# Autodesk Inventor assembly: Super Gantry
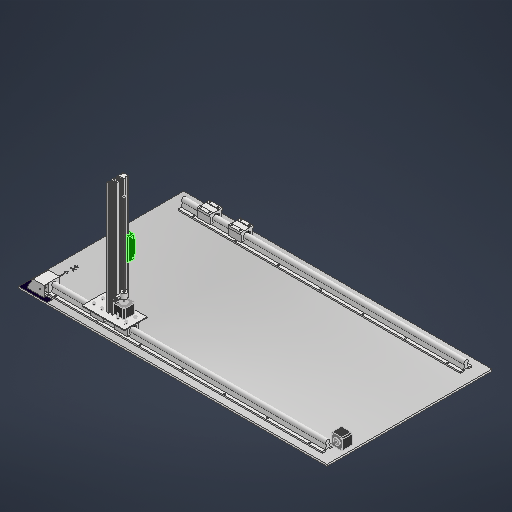
[picture p0: Inventor's stored thumbnail of the model, 512x512]
Saved by Autodesk Inventor 2025.1 (Build 291241000, 241)
## iProperties
Created: 2025-01-22
Part Number: Super Gantry
Document SubType Name: Assembly
Designer: jerem
Author: jerem
## Documents named in this file (3)
- C:\Users\jerem\Documents\GitHub\Perovskite-Automated-Synthesis-System\CAD\Gantry\Super Gantry.iam
- C:\Users\jerem\Documents\GitHub\Perovskite-Automated-Synthesis-System\CAD\Gantry\X Axis.iam
- C:\Users\jerem\Documents\GitHub\Perovskite-Automated-Synthesis-System\CAD\Gantry\Z Axis.iam
## Components (2 placed, 2 different names)
1. X Axis:1 [sub-assembly] — Mate:1, Mate:2, Mate:3, Mate:4, Mate:5
2. Z Axis:1 [sub-assembly] — Mate:1, Mate:2, Mate:3, Mate:4, Mate:5
## Relationships (5: Mate 5)
- Mate:1: X Axis:1 ↔ Z Axis:1
- Mate:2: X Axis:1 ↔ Z Axis:1
- Mate:3: X Axis:1 ↔ Z Axis:1
- Mate:4: X Axis:1 ↔ Z Axis:1
- Mate:5: X Axis:1 ↔ Z Axis:1
